# Autodesk Inventor assembly: BottomRobot
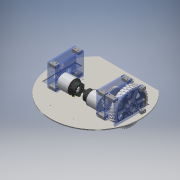
[picture p0: Inventor's stored thumbnail of the model, 180x180]
Saved by Autodesk Inventor 2019 (Build 230136000, 136)
## iProperties
Created: 2020-03-02
Part Number: BottomRobot
Document SubType Name: Assembly
Designer: james
Author: james
## Documents named in this file (4)
- F:\JimsRobot\FIRSTRobots\Design\TornadoPlatypus\BottomRobot.iam
- F:\JimsRobot\FIRSTRobots\Design\TornadoPlatypus\BottomPlate.ipt
- F:\JimsRobot\FIRSTRobots\Design\TornadoPlatypus\MotorLeft.iam
- F:\JimsRobot\FIRSTRobots\Design\TornadoPlatypus\MotorRight.iam
## Components (3 placed, 3 different names)
1. BottomPlate:1 — Mate:1, Mate:2, Mate:3, Mate:4, Mate:5
2. MotorLeft:1 [sub-assembly] — Mate:1, Mate:3, Mate:5
3. MotorRight:1 [sub-assembly] — Mate:2, Mate:4
## Relationships (5: Mate 5)
- Mate:1: BottomPlate:1 ↔ MotorLeft:1
- Mate:2: BottomPlate:1 ↔ MotorRight:1
- Mate:3: BottomPlate:1 ↔ MotorLeft:1
- Mate:4: BottomPlate:1 ↔ MotorRight:1
- Mate:5: BottomPlate:1 ↔ MotorLeft:1
